# Autodesk Inventor assembly: 6P Sprocket
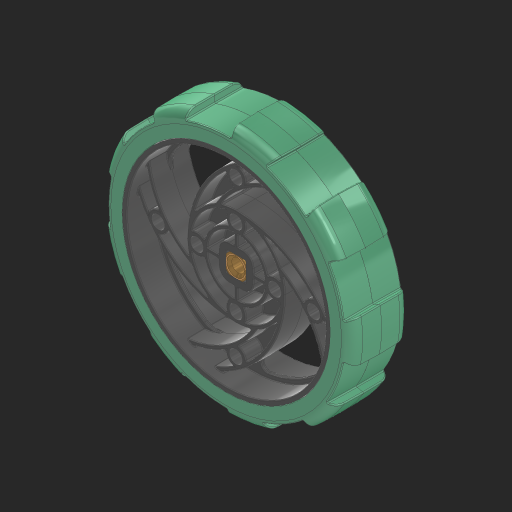
[picture p0: Inventor's stored thumbnail of the model, 512x512]
Saved by Autodesk Inventor 2023 (Build 270158000, 158)
## iProperties
Created: 2022-08-02
Part Number: 6P Sprocket
Document SubType Name: Assembly
Designer: ylu12
Author: ylu12
## Documents named in this file (4)
- C:\Users\ylu12\Documents\GitHub\VEX-CAD-Inventor\Motion\Wheels\Traction Wheel\3.25 Traction, Circle.iam
- C:\Users\ylu12\Documents\GitHub\VEX-CAD-Inventor\Motion\Wheels\Reference Files\3.25 Traction.ipt
- C:\Users\ylu12\Documents\GitHub\VEX-CAD-Inventor\Motion\HS Shaft Adapter Circle.ipt
- C:\Users\ylu12\Documents\GitHub\VEX-CAD-Inventor\Motion\Wheels\Traction Wheel.iam
## Components (2 placed, 2 different names)
1. 3.25 Traction — Flush:4, Mate:7, Mate:8
2. Circle — Mate:32, Mate:33, Flush:10
## Relationships (6: Mate 4, Flush 2)
- Flush:4: 3.25 Traction
- Mate:7: 3.25 Traction
- Mate:8: 3.25 Traction
- Mate:32: Circle
- Mate:33: Circle
- Flush:10 (6.35 mm): Circle
## Named parameters: Thickness = 8.255 mm
